# Autodesk Inventor assembly: Assembly1
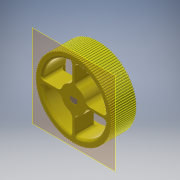
[picture p0: Inventor's stored thumbnail of the model, 180x180]
Saved by Autodesk Inventor 2019 (Build 230136000, 136)
## iProperties
Created: 2019-09-12
Part Number: Assembly1
Document SubType Name: Assembly
Designer: assman
Author: assman
## Documents named in this file (3)
- D:\Inventor\Projects\ArduSpinner\Assembly1.iam
- D:\Inventor\Projects\ArduSpinner\wheel.ipt
- D:\Inventor\Projects\ArduSpinner\encoder.ipt
## Components (2 placed, 2 different names)
1. wheel:1 — Rotational:1
2. encoder:1 — Rotational:1
## Relationships (1: RevoluteJoint 1)
- Rotational:1 [RevoluteJoint]: wheel:1 ↔ encoder:1
